# Autodesk Inventor assembly: Assembly1
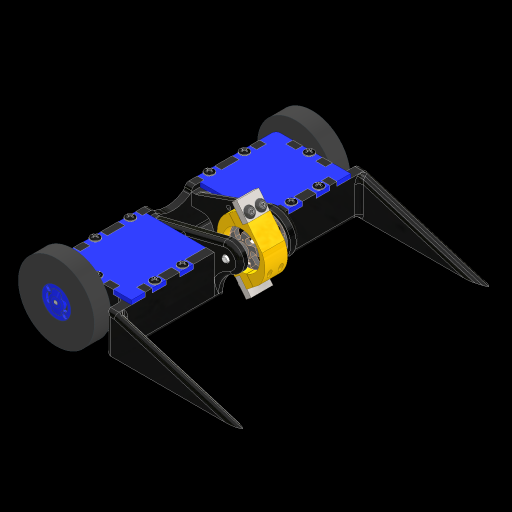
[picture p0: Inventor's stored thumbnail of the model, 512x512]
Saved by Autodesk Inventor 2023 (Build 270158000, 158)
## iProperties
Created: 2023-07-31
Part Number: Assembly1
Document SubType Name: Assembly
Designer: tandu
Mass: 344.46 g
Surface Area: 1075.14 cm^2
Volume: 242.159 cm^3
Density: 1.42245 g/cm^3
Author: tandu
## Documents named in this file (14)
- C:\Users\tandu\Documents\GrabCAD\Combat Robot Kits\To Sell\2WD Vertical Reach\Inventor CAD Source Files\Assembly1.iam
- C:\Users\tandu\Documents\GrabCAD\Combat Robot Kits\To Sell\2WD Vertical Reach\Inventor CAD Source Files\Chassis.ipt
- C:\Users\tandu\Documents\GrabCAD\Combat Robot Kits\To Sell\2WD Vertical Reach\Inventor CAD Source Files\BearingUpright.ipt
- C:\Users\tandu\Documents\GrabCAD\Combat Robot Kits\To Sell\2WD Vertical Reach\Inventor CAD Source Files\MotorUpright.ipt
- C:\Users\tandu\Documents\GrabCAD\Combat Robot Kits\To Sell\2WD Vertical Reach\Inventor CAD Source Files\2 25 in x 0 50 in FT Wheel.ipt
- C:\Users\tandu\Documents\GrabCAD\Combat Robot Kits\To Sell\2WD Vertical Reach\Inventor CAD Source Files\300mAh 3S Lumenier Battery Mockup.ipt
- C:\Users\tandu\Documents\GrabCAD\Combat Robot Kits\To Sell\2WD Vertical Reach\Inventor CAD Source Files\FingerTech_Silver_Spark_223350.ipt
- C:\Users\tandu\Documents\GrabCAD\Combat Robot Kits\To Sell\2WD Vertical Reach\Inventor CAD Source Files\ClampDrum\ClampDrumAssembly.iam
- C:\Users\tandu\Documents\GrabCAD\Combat Robot Kits\To Sell\2WD Vertical Reach\Inventor CAD Source Files\ClampDrum\D2822 Motor.ipt
- C:\Users\tandu\Documents\Inventor\Content Center Files\R2023\en-US\ISO 10642(2)\ISO 10642  - M3  x  8.ipt
- C:\Users\tandu\Documents\GrabCAD\Combat Robot Kits\To Sell\2WD Vertical Reach\Inventor CAD Source Files\4 x 8 x 8 mm Needle Bearing Mockup.ipt
- C:\Users\tandu\Documents\GrabCAD\Combat Robot Kits\To Sell\2WD Vertical Reach\Inventor CAD Source Files\TopPlate.ipt
- C:\Users\tandu\Documents\GrabCAD\Combat Robot Kits\To Sell\2WD Vertical Reach\Inventor CAD Source Files\TopPlate_MIR.ipt
- C:\Users\tandu\Documents\GrabCAD\Combat Robot Kits\To Sell\2WD Vertical Reach\Inventor CAD Source Files\90417A126_Phillips Rounded Head Thread-Forming Screws.ipt
## Components (33 placed, 13 different names)
1. Chassis:1 — Insert:1, Mate:1, Insert:2, Mate:2, Mate:3, Mate:4, Mate:5, Insert:3, Insert:4, Insert:5, Insert:6, Insert:7, Insert:8, Insert:17, Insert:18, Insert:29, Insert:30, Insert:31, Insert:32, Insert:33, Insert:34
2. BearingUpright:1 — Insert:5, Insert:6, Symmetry:1
3. MotorUpright:1 — Insert:7, Insert:8, Insert:9, Insert:10, Insert:12, Insert:13, Insert:14, Insert:15, Symmetry:1
4. 2 25 in x 0 50 in FT Wheel:1 — Insert:3
5. 300mAh 3S Lumenier Battery Mockup:1 — Mate:3, Mate:4, Mate:5
6. FingerTech_Silver_Spark_223350:1 — Insert:1, Mate:1
7. 2 25 in x 0 50 in FT Wheel:2 — Insert:4
8. FingerTech_Silver_Spark_223350:2 — Insert:2, Mate:2
9. ClampDrumAssembly:1 [sub-assembly] — Insert:11
10. D2822 Motor:1 — Insert:9, Insert:10, Insert:11, Insert:16
11. DIN EN ISO 10642 M3  x  8:1 — Insert:12
12. DIN EN ISO 10642 M3  x  8:2 — Insert:13
13. DIN EN ISO 10642 M3  x  8:3 — Insert:14
14. DIN EN ISO 10642 M3  x  8:4 — Insert:15
15. 4 x 8 x 8 mm Needle Bearing Mockup:1 — Insert:16
16. TopPlate:1 — Insert:17, Insert:18, Insert:19, Insert:20, Insert:21, Insert:22, Insert:23
17. TopPlate_MIR:1 — Insert:24, Insert:25, Insert:26, Insert:27, Insert:28
18. 90417A126_Phillips Rounded Head Thread-Forming Screws:1 — Insert:22
19. 90417A126_Phillips Rounded Head Thread-Forming Screws:2 — Insert:23
20. 90417A126_Phillips Rounded Head Thread-Forming Screws:3 — Insert:19
21. 90417A126_Phillips Rounded Head Thread-Forming Screws:4 — Insert:20
22. 90417A126_Phillips Rounded Head Thread-Forming Screws:5 — Insert:21
23. 90417A126_Phillips Rounded Head Thread-Forming Screws:6 — Insert:24
24. 90417A126_Phillips Rounded Head Thread-Forming Screws:7 — Insert:25
25. 90417A126_Phillips Rounded Head Thread-Forming Screws:8 — Insert:26
26. 90417A126_Phillips Rounded Head Thread-Forming Screws:9 — Insert:28
27. 90417A126_Phillips Rounded Head Thread-Forming Screws:10 — Insert:27
28. 90417A126_Phillips Rounded Head Thread-Forming Screws:11 — Insert:32
29. 90417A126_Phillips Rounded Head Thread-Forming Screws:12 — Insert:30
30. 90417A126_Phillips Rounded Head Thread-Forming Screws:13 — Insert:31
31. 90417A126_Phillips Rounded Head Thread-Forming Screws:14 — Insert:29
32. 90417A126_Phillips Rounded Head Thread-Forming Screws:15 — Insert:33
33. 90417A126_Phillips Rounded Head Thread-Forming Screws:16 — Insert:34
## Relationships (40: Insert 34, Mate 5, Symmetry 1)
- Insert:1: Chassis:1 ↔ FingerTech_Silver_Spark_223350:1
- Mate:1: Chassis:1 ↔ FingerTech_Silver_Spark_223350:1
- Insert:2: Chassis:1 ↔ FingerTech_Silver_Spark_223350:2
- Mate:2: Chassis:1 ↔ FingerTech_Silver_Spark_223350:2
- Mate:3: Chassis:1 ↔ 300mAh 3S Lumenier Battery Mockup:1
- Mate:4: Chassis:1 ↔ 300mAh 3S Lumenier Battery Mockup:1
- Mate:5: Chassis:1 ↔ 300mAh 3S Lumenier Battery Mockup:1
- Insert:3: Chassis:1 ↔ 2 25 in x 0 50 in FT Wheel:1
- Insert:4: Chassis:1 ↔ 2 25 in x 0 50 in FT Wheel:2
- Insert:5: Chassis:1 ↔ BearingUpright:1
- Insert:6: Chassis:1 ↔ BearingUpright:1
- Insert:7: Chassis:1 ↔ MotorUpright:1
- Insert:8: Chassis:1 ↔ MotorUpright:1
- Insert:9: MotorUpright:1 ↔ D2822 Motor:1
- Insert:10: MotorUpright:1 ↔ D2822 Motor:1
- Insert:11: ClampDrumAssembly:1 ↔ D2822 Motor:1
- Insert:12: MotorUpright:1 ↔ DIN EN ISO 10642 M3  x  8:1
- Insert:13: MotorUpright:1 ↔ DIN EN ISO 10642 M3  x  8:2
- Insert:14: MotorUpright:1 ↔ DIN EN ISO 10642 M3  x  8:3
- Insert:15: MotorUpright:1 ↔ DIN EN ISO 10642 M3  x  8:4
- Insert:16: D2822 Motor:1 ↔ 4 x 8 x 8 mm Needle Bearing Mockup:1
- Insert:17: Chassis:1 ↔ TopPlate:1
- Insert:18: Chassis:1 ↔ TopPlate:1
- Symmetry:1: BearingUpright:1 ↔ MotorUpright:1
- Insert:19: TopPlate:1 ↔ 90417A126_Phillips Rounded Head Thread-Forming Screws:3
- Insert:20: TopPlate:1 ↔ 90417A126_Phillips Rounded Head Thread-Forming Screws:4
- Insert:21: TopPlate:1 ↔ 90417A126_Phillips Rounded Head Thread-Forming Screws:5
- Insert:22: TopPlate:1 ↔ 90417A126_Phillips Rounded Head Thread-Forming Screws:1
- Insert:23: TopPlate:1 ↔ 90417A126_Phillips Rounded Head Thread-Forming Screws:2
- Insert:24: TopPlate_MIR:1 ↔ 90417A126_Phillips Rounded Head Thread-Forming Screws:6
- Insert:25: TopPlate_MIR:1 ↔ 90417A126_Phillips Rounded Head Thread-Forming Screws:7
- Insert:26: TopPlate_MIR:1 ↔ 90417A126_Phillips Rounded Head Thread-Forming Screws:8
- Insert:27: TopPlate_MIR:1 ↔ 90417A126_Phillips Rounded Head Thread-Forming Screws:10
- Insert:28: TopPlate_MIR:1 ↔ 90417A126_Phillips Rounded Head Thread-Forming Screws:9
- Insert:29: Chassis:1 ↔ 90417A126_Phillips Rounded Head Thread-Forming Screws:14
- Insert:30: Chassis:1 ↔ 90417A126_Phillips Rounded Head Thread-Forming Screws:12
- Insert:31: Chassis:1 ↔ 90417A126_Phillips Rounded Head Thread-Forming Screws:13
- Insert:32: Chassis:1 ↔ 90417A126_Phillips Rounded Head Thread-Forming Screws:11
- Insert:33: Chassis:1 ↔ 90417A126_Phillips Rounded Head Thread-Forming Screws:15
- Insert:34: Chassis:1 ↔ 90417A126_Phillips Rounded Head Thread-Forming Screws:16
